# Autodesk Inventor assembly: H-Shaped-Assembly
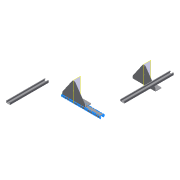
[picture p0: Inventor's stored thumbnail of the model, 180x180]
Saved by Autodesk Inventor 2015 (Build 190159000, 159)
## iProperties
Created: 2015-01-24
Part Number: H-Shaped-Assembly
Document SubType Name: Assembly
Designer: Peter
Author: Peter
## Documents named in this file (4)
- T:\FILES\FIRST-Team-1719-CAD-Team\2015 Robot CAD\Two Lifters and Lifter Super Structure\Lifter Super Structure\Tower\H-Shaped-Assembly\H-Shaped-Assembly.iam
- T:\FILES\FIRST-Team-1719-CAD-Team\2015 Robot CAD\Two Lifters and Lifter Super Structure\Lifter Super Structure\Tower\H-Shaped-Assembly\Horizontal-Center-Brace-H-Shape.ipt
- T:\FILES\FIRST-Team-1719-CAD-Team\2015 Robot CAD\Two Lifters and Lifter Super Structure\Lifter Super Structure\Tower\H-Shaped-Assembly\Horizontal-Unistrut-Tower-Connector-19-25.ipt
- T:\FILES\FIRST-Team-1719-CAD-Team\2015 Robot CAD\Two Lifters and Lifter Super Structure\Lifter Super Structure\Tower\H-Shaped-Assembly\Horizontal-Unistrut-Tower-Connector-15.ipt
## Components (5 placed, 3 different names)
1. Horizontal-Center-Brace-H-Shape:1
2. Horizontal-Unistrut-Tower-Connector-19-25:1
3. Horizontal-Unistrut-Tower-Connector-15:1 — Mate:1, Flush:1
4. Horizontal-Center-Brace-H-Shape:2 — Mate:1, Flush:1
5. Horizontal-Unistrut-Tower-Connector-15:2
## Relationships (2: Mate 1, Flush 1)
- Mate:1: Horizontal-Unistrut-Tower-Connector-15:1 ↔ Horizontal-Center-Brace-H-Shape:2
- Flush:1: Horizontal-Unistrut-Tower-Connector-15:1 ↔ Horizontal-Center-Brace-H-Shape:2
